# Autodesk Inventor assembly: Сборка_KIA_ProCeed
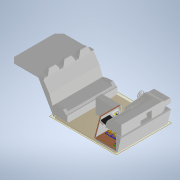
[picture p0: Inventor's stored thumbnail of the model, 180x180]
Saved by Autodesk Inventor 2021.2 (Build 252289000, 289)
## iProperties
Created: 2021-10-11
Part Number: Сборка_KIA_ProCeed
Document SubType Name: Assembly
Designer: Surflay
Author: Surflay
## Documents named in this file (22)
- C:\Users\Surflay\OneDrive\Рабочий стол\Modeling\Power_supply_Car_Model\Сборка_KIA_ProCeed.iam
- C:\Users\Surflay\OneDrive\Рабочий стол\Modeling\Power_supply_Car_Model\ДИ 00.00.02.ipt
- C:\Users\Surflay\OneDrive\Рабочий стол\Modeling\Power_supply_Car_Model\ДИ 00.00.01.ipt
- C:\Users\Surflay\OneDrive\Рабочий стол\Modeling\Power_supply_Car_Model\ДИ 00.00.03.ipt
- C:\Users\Surflay\OneDrive\Рабочий стол\Modeling\Power_supply_Car_Model\ДИ 00.00.03_MIR.ipt
- C:\Users\Surflay\OneDrive\Рабочий стол\Modeling\Power_supply_Car_Model\Деталь4.ipt
- C:\Users\Surflay\OneDrive\Рабочий стол\Modeling\Power_supply_Car_Model\Деталь4_MIR.ipt
- C:\Users\Surflay\OneDrive\Рабочий стол\Modeling\Power_supply_Car_Model\ДИ 00.00.06.ipt
- C:\Users\Surflay\OneDrive\Рабочий стол\Modeling\Power_supply_Car_Model\ДИ 00.00.07.ipt
- C:\Users\Surflay\OneDrive\Рабочий стол\Modeling\Power_supply_Car_Model\Деталь8.ipt
- C:\Users\Surflay\OneDrive\Рабочий стол\Modeling\Power_supply_Car_Model\ДИ 00.00.08.ipt
- C:\Users\Surflay\OneDrive\Рабочий стол\Modeling\Power_supply_Car_Model\ДИ 00.00.09.ipt
- C:\Users\Surflay\OneDrive\Рабочий стол\Modeling\Power_supply_Car_Model\ДИ 00.00.10.ipt
- C:\Users\Surflay\OneDrive\Рабочий стол\Modeling\Power_supply_Car_Model\ДИ 00.00.11.ipt
- C:\Users\Surflay\OneDrive\Рабочий стол\Modeling\Power_supply_Car_Model\ДИ 00.00.12.ipt
- C:\Users\Surflay\OneDrive\Рабочий стол\Modeling\Power_supply_Car_Model\Интвертор.ipt
- C:\Users\Surflay\OneDrive\Рабочий стол\Modeling\Power_supply_Car_Model\Клемники винтовые.ipt
- C:\Users\Surflay\OneDrive\Рабочий стол\Modeling\Power_supply_Car_Model\Преобразователь напряжения.ipt
- C:\Users\Surflay\OneDrive\Рабочий стол\Modeling\Power_supply_Car_Model\Сборка_KIA_ProCeed\AIP\Провода и кабели\Сборка_KIA_ProCeed.Прокладка кабелей1.iam
- C:\Users\Surflay\OneDrive\Рабочий стол\Modeling\Power_supply_Car_Model\Задние_кресла.ipt
- C:\Users\Surflay\OneDrive\Рабочий стол\Modeling\Power_supply_Car_Model\Руль.ipt
- C:\Users\Surflay\OneDrive\Рабочий стол\Modeling\Power_supply_Car_Model\Кранштейн сервомоторов.ipt
## Components (24 placed, 21 different names)
1. ДИ 00.00.02:1 — Совмещение:1, Совмещение:2, Совмещение:3, Заподлицо:14, Заподлицо:15
2. ДИ 00.00.01:1 — Совмещение:1, Совмещение:2, Совмещение:3, Совмещение:4, Совмещение:5, Совмещение:6, Совмещение:7, Совмещение:8, Совмещение:9, Заподлицо:1, Совмещение:10, Заподлицо:2, Заподлицо:3, Заподлицо:4, Заподлицо:5, Заподлицо:11, Заподлицо:12, Заподлицо:13, Заподлицо:16, Заподлицо:17
3. ДИ 00.00.03:1 — Совмещение:4, Совмещение:5, Совмещение:6
4. ДИ 00.00.03_MIR:1 — Совмещение:7, Совмещение:8, Совмещение:9, Совмещение:11, Совмещение:12
5. Деталь4:1 — Заподлицо:1
6. Деталь4_MIR:1 — Совмещение:10, Совмещение:11, Совмещение:12
7. ДИ 00.00.06:1 — Заподлицо:2
8. ДИ 00.00.07:1 — Заподлицо:3
9. Деталь8:1 — Заподлицо:4
10. ДИ 00.00.08:1 — Заподлицо:5, Заподлицо:6, Совмещение:13, Совмещение:14, Заподлицо:7, Совмещение:19, Совмещение:20, Заподлицо:9, Совмещение:26, Совмещение:27, Совмещение:28, Совмещение:29, Совмещение:30, Заподлицо:10
11. ДИ 00.00.09:1 — Заподлицо:6, Совмещение:13, Совмещение:24, Совмещение:25, Заподлицо:8
12. ДИ 00.00.10:1 — Совмещение:14, Совмещение:16, Совмещение:23
13. ДИ 00.00.11:1 — Совмещение:24, Совмещение:25
14. ДИ 00.00.10:2 — Совмещение:18, Совмещение:19, Совмещение:22, Совмещение:23
15. ДИ 00.00.10:3 — Совмещение:20, Совмещение:21, Совмещение:22
16. ДИ 00.00.12:1 — Заподлицо:7, Совмещение:16, Совмещение:18, Совмещение:21
17. Интвертор:1 — Заподлицо:8
18. Клемники винтовые:1 — Заподлицо:9, Совмещение:26, Совмещение:27, Совмещение:28
19. Клемники винтовые:2 — Совмещение:29, Совмещение:30
20. Преобразователь напряжения:1 — Заподлицо:10
21. Прокладка кабелей1 [sub-assembly]
22. Задние_кресла:1 — Заподлицо:11, Заподлицо:12, Заподлицо:13
23. Руль:1 — Заподлицо:14, Заподлицо:15
24. Кранштейн сервомоторов:1 — Заподлицо:16, Заподлицо:17
## Relationships (45: Mate 28, Flush 17)
- Совмещение:1 [Mate]: ДИ 00.00.02:1 ↔ ДИ 00.00.01:1
- Совмещение:2 [Mate]: ДИ 00.00.02:1 ↔ ДИ 00.00.01:1
- Совмещение:3 [Mate]: ДИ 00.00.02:1 ↔ ДИ 00.00.01:1
- Совмещение:4 [Mate]: ДИ 00.00.01:1 ↔ ДИ 00.00.03:1
- Совмещение:5 [Mate]: ДИ 00.00.01:1 ↔ ДИ 00.00.03:1
- Совмещение:6 [Mate]: ДИ 00.00.01:1 ↔ ДИ 00.00.03:1
- Совмещение:7 [Mate]: ДИ 00.00.01:1 ↔ ДИ 00.00.03_MIR:1
- Совмещение:8 [Mate]: ДИ 00.00.01:1 ↔ ДИ 00.00.03_MIR:1
- Совмещение:9 [Mate]: ДИ 00.00.01:1 ↔ ДИ 00.00.03_MIR:1
- Заподлицо:1 [Flush]: ДИ 00.00.01:1 ↔ Деталь4:1
- Совмещение:10 [Mate]: ДИ 00.00.01:1 ↔ Деталь4_MIR:1
- Совмещение:11 [Mate]: ДИ 00.00.03_MIR:1 ↔ Деталь4_MIR:1
- Совмещение:12 [Mate]: ДИ 00.00.03_MIR:1 ↔ Деталь4_MIR:1
- Заподлицо:2 [Flush]: ДИ 00.00.01:1 ↔ ДИ 00.00.06:1
- Заподлицо:3 [Flush]: ДИ 00.00.01:1 ↔ ДИ 00.00.07:1
- Заподлицо:4 [Flush]: ДИ 00.00.01:1 ↔ Деталь8:1
- Заподлицо:5 [Flush]: ДИ 00.00.01:1 ↔ ДИ 00.00.08:1
- Заподлицо:6 [Flush]: ДИ 00.00.08:1 ↔ ДИ 00.00.09:1
- Совмещение:13 [Mate]: ДИ 00.00.08:1 ↔ ДИ 00.00.09:1
- Совмещение:14 [Mate]: ДИ 00.00.08:1 ↔ ДИ 00.00.10:1
- Заподлицо:7 [Flush]: ДИ 00.00.08:1 ↔ ДИ 00.00.12:1
- Совмещение:16 [Mate] (5 mm): ДИ 00.00.10:1 ↔ ДИ 00.00.12:1
- Совмещение:18 [Mate] (5 mm): ДИ 00.00.10:2 ↔ ДИ 00.00.12:1
- Совмещение:19 [Mate]: ДИ 00.00.08:1 ↔ ДИ 00.00.10:2
- Совмещение:20 [Mate]: ДИ 00.00.08:1 ↔ ДИ 00.00.10:3
- Совмещение:21 [Mate] (5 mm): ДИ 00.00.10:3 ↔ ДИ 00.00.12:1
- Совмещение:22 [Mate] (1 mm): ДИ 00.00.10:2 ↔ ДИ 00.00.10:3
- Совмещение:23 [Mate] (1 mm): ДИ 00.00.10:1 ↔ ДИ 00.00.10:2
- Совмещение:24 [Mate]: ДИ 00.00.09:1 ↔ ДИ 00.00.11:1
- Совмещение:25 [Mate]: ДИ 00.00.09:1 ↔ ДИ 00.00.11:1
- Заподлицо:8 [Flush]: ДИ 00.00.09:1 ↔ Интвертор:1
- Заподлицо:9 [Flush]: ДИ 00.00.08:1 ↔ Клемники винтовые:1
- Совмещение:26 [Mate]: ДИ 00.00.08:1 ↔ Клемники винтовые:1
- Совмещение:27 [Mate]: ДИ 00.00.08:1 ↔ Клемники винтовые:1
- Совмещение:28 [Mate]: ДИ 00.00.08:1 ↔ Клемники винтовые:1
- Совмещение:29 [Mate]: ДИ 00.00.08:1 ↔ Клемники винтовые:2
- Совмещение:30 [Mate]: ДИ 00.00.08:1 ↔ Клемники винтовые:2
- Заподлицо:10 [Flush]: ДИ 00.00.08:1 ↔ Преобразователь напряжения:1
- Заподлицо:11 [Flush]: ДИ 00.00.01:1 ↔ Задние_кресла:1
- Заподлицо:12 [Flush]: ДИ 00.00.01:1 ↔ Задние_кресла:1
- Заподлицо:13 [Flush]: ДИ 00.00.01:1 ↔ Задние_кресла:1
- Заподлицо:14 [Flush]: ДИ 00.00.02:1 ↔ Руль:1
- Заподлицо:15 [Flush]: ДИ 00.00.02:1 ↔ Руль:1
- Заподлицо:16 [Flush]: ДИ 00.00.01:1 ↔ Кранштейн сервомоторов:1
- Заподлицо:17 [Flush]: ДИ 00.00.01:1 ↔ Кранштейн сервомоторов:1
